# Autodesk Inventor assembly: GripperMount
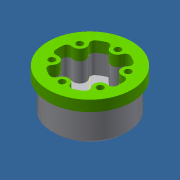
[picture p0: Inventor's stored thumbnail of the model, 180x180]
Saved by Autodesk Inventor 2016 (Build 200138000, 138)
## iProperties
Created: 2015-09-10
Part Number: GripperMount
Material: Generisch
Document SubType Name: Assembly
Designer: 4ndreas
Mass: 10.9804 g
Surface Area: 82.4709 cm^2
Volume: 10.3589 cm^3
Density: 1.06 g/cm^3
Author: 4ndreas
## Documents named in this file (3)
- C:\Users\4ndreas\Documents\Inventor\RobotARM v2\v4\GripperMount.iam
- C:\Users\4ndreas\Documents\Inventor\RobotARM v2\v4\GripperMount.ipt
- C:\Users\4ndreas\Documents\Inventor\RobotARM v2\v4\GripperMountPlate.ipt
## Components (2 placed, 2 different names)
1. GripperMount:1 — Fluchtend:1, Fluchtend:2, Fluchtend:3, Passend:1, Fluchtend:4
2. GripperMountPlate:1 — Fluchtend:4
## Relationships (5: Flush 4, Mate 1)
- Fluchtend:1 [Flush]: GripperMount:1
- Fluchtend:2 [Flush]: GripperMount:1
- Fluchtend:3 [Flush]: GripperMount:1
- Passend:1 [Mate]: GripperMount:1
- Fluchtend:4 [Flush]: GripperMount:1 ↔ GripperMountPlate:1
